# Autodesk Inventor assembly: Odom Pod
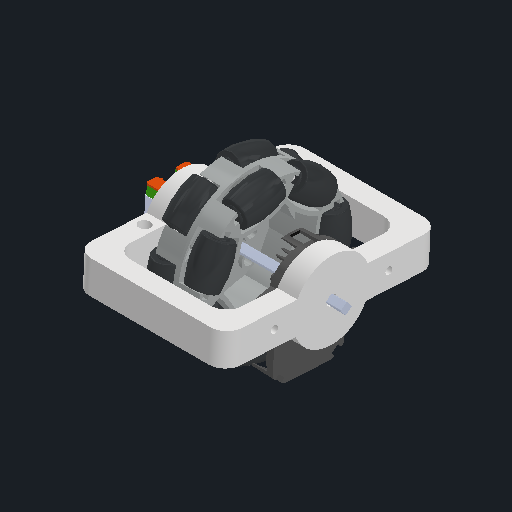
[picture p0: Inventor's stored thumbnail of the model, 512x512]
Saved by Autodesk Inventor 2025.1 (Build 291241000, 241)
## iProperties
Created: 2024-12-18
Part Number: Odom Pod
Document SubType Name: Assembly
Designer: Juan
Author: Juan
## Documents named in this file (12)
- C:\Users\Juanl\Documents\GitHub\ATUM-V5RC-High-Stakes-CAD\Robot\Subassemblies\Odom Pod.iam
- C:\Users\Juanl\Documents\GitHub\ATUM-V5RC-High-Stakes-CAD\Odometers_Collin\IQ_OMNI.iam
- C:\Users\Juanl\Documents\GitHub\ATUM-V5RC-High-Stakes-CAD\Odometers_Collin\Linear Rail Files\Carriage-LWL7B\Carriage-LWL7B\Carriage-LWL7B.ipt
- C:\Users\Juanl\Documents\GitHub\ATUM-V5RC-High-Stakes-CAD\Odometers_Collin\Linear_Odom.ipt
- C:\Users\Juanl\Documents\GitHub\ATUM-V5RC-High-Stakes-CAD\VEX-CAD-Inventor\Motion\Insert Circle.ipt
- C:\Users\Juanl\Documents\GitHub\ATUM-V5RC-High-Stakes-CAD\VEX-CAD-Inventor\Motion\Spacers\Washer Teflon\TWasher .375 OD x .06250.ipt
- C:\Users\Juan\Documents\GitHub\ATUM-VRC-High-Stakes-CAD\VEX-CAD-Inventor\Motion\Spacers\Washer Teflon.ipt
- C:\Users\Juanl\Documents\GitHub\ATUM-V5RC-High-Stakes-CAD\VEX-CAD-Inventor\Motion\Spacers\Spacer Nylon .375 OD\NSpacer .375 OD x .125.ipt
- C:\Users\Juan\Documents\GitHub\ATUM-VRC-High-Stakes-CAD\VEX-CAD-Inventor\Motion\Spacers\Spacer Nylon .375 OD.ipt
- C:\Users\Juanl\Documents\GitHub\ATUM-V5RC-High-Stakes-CAD\VEX-CAD-Inventor\Motion\Shaft LS\Shaft LS\Shaft LS 2.5.ipt
- C:\Users\Juan\Documents\GitHub\ATUM-VRC-High-Stakes-CAD\VEX-CAD-Inventor\Motion\Shaft LS\Shaft LS.ipt
- C:\Users\Juanl\Documents\GitHub\ATUM-V5RC-High-Stakes-CAD\Encoder_Files\AMT-102-Wide-Base-REV-J.ipt
## Components (9 placed, 8 different names)
1. IQ_OMNI:1 [sub-assembly]
2. Carriage-LWL7B:1
3. Linear_Odom:1
4. Insert Circle:1
5. TWasher .375 OD x .06250:1
6. TWasher .375 OD x .06250:2
7. NSpacer .375 OD x .125:1
8. Shaft LS 2.5:1
9. AMT-102-Wide-Base-REV-J:1
## Relationships (21: Mate 21)
- [Mate] (0.0762 mm): Linear_Odom:1 ↔ Insert Circle:1
- [Mate] (0.0762 mm): Linear_Odom:1 ↔ Insert Circle:1
- [Mate]: Linear_Odom:1 ↔ Insert Circle:1
- [Mate]: Carriage-LWL7B:1 ↔ Linear_Odom:1
- [Mate]: Carriage-LWL7B:1 ↔ Linear_Odom:1
- [Mate]: Carriage-LWL7B:1 ↔ Linear_Odom:1
- [Mate]: Insert Circle:1 ↔ TWasher .375 OD x .06250:1
- [Mate]: Insert Circle:1 ↔ TWasher .375 OD x .06250:1
- [Mate]: TWasher .375 OD x .06250:1 ↔ NSpacer .375 OD x .125:1
- [Mate]: TWasher .375 OD x .06250:1 ↔ NSpacer .375 OD x .125:1
- [Mate]: TWasher .375 OD x .06250:2 ↔ NSpacer .375 OD x .125:1
- [Mate]: TWasher .375 OD x .06250:2 ↔ NSpacer .375 OD x .125:1
- [Mate]: Linear_Odom:1 ↔ Shaft LS 2.5:1
- [Mate]: TWasher .375 OD x .06250:2 ↔ Shaft LS 2.5:1
- [Mate]: Linear_Odom:1 ↔ Shaft LS 2.5:1
- [Mate]: IQ_OMNI:1 ↔ TWasher .375 OD x .06250:2
- [Mate]: IQ_OMNI:1 ↔ Shaft LS 2.5:1
- [Mate]: IQ_OMNI:1 ↔ Shaft LS 2.5:1
- [Mate]: Linear_Odom:1 ↔ AMT-102-Wide-Base-REV-J:1
- [Mate]: Linear_Odom:1 ↔ AMT-102-Wide-Base-REV-J:1
- [Mate]: Linear_Odom:1 ↔ AMT-102-Wide-Base-REV-J:1
## Named parameters: d1954_d1934 = 0 mm, d1955_d1924 = 0 mm, d1956_d1925 = 0 mm, d1957_d1926 = 0 mm, d1958_d1914 = 0.0762 mm, d1959_d1915 = 0.0762 mm, d1960_d1916 = 0 mm, d1961_d1917 = 0 mm, d1962_d1918 = 0 mm, d1963_d1919 = 0 mm, d1964_d1921 = 0 mm, d1965_d1922 = 0 mm, d1966_d1923 = 0 mm
